# Autodesk Inventor assembly: Draft_01
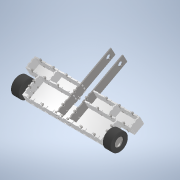
[picture p0: Inventor's stored thumbnail of the model, 180x180]
Saved by Autodesk Inventor 2021 (Build 250183000, 183)
## iProperties
Created: 2021-03-05
Part Number: Draft_01
Document SubType Name: Assembly
Designer: M3rob
Mass: 48019.6 g
Surface Area: 29850.8 cm^2
Volume: 13431.3 cm^3
Density: 3.57521 g/cm^3
Author: M3rob
## Documents named in this file (13)
- C:\Users\M3rob\Documents\GrabCAD\FireBird 250 Pound Gaming Machine\Drafts\FrameDrafts\Draft_01\Draft_01.iam
- C:\Users\M3rob\Documents\GrabCAD\FireBird 250 Pound Gaming Machine\Drafts\FrameDrafts\Draft_01\BackWallFrame.ipt
- C:\Users\M3rob\Documents\GrabCAD\FireBird 250 Pound Gaming Machine\Drafts\FrameDrafts\Draft_01\DriveFrame.ipt
- C:\Users\M3rob\Documents\GrabCAD\FireBird 250 Pound Gaming Machine\Drafts\FrameDrafts\Draft_01\NeckFrame.ipt
- C:\Users\M3rob\Documents\GrabCAD\FireBird 250 Pound Gaming Machine\Drafts\FrameDrafts\Draft_01\FrontFrame.ipt
- C:\Users\M3rob\Documents\GrabCAD\FireBird 250 Pound Gaming Machine\Drafts\FrameDrafts\Draft_01\SmallSideFrame.ipt
- C:\Users\M3rob\Documents\GrabCAD\FireBird 250 Pound Gaming Machine\Drafts\FrameDrafts\Draft_01\AluminumTopPlate.ipt
- C:\Users\M3rob\Documents\Inventor\Content Center Files\R2021\en-US\AS 2465(2)\AS 2465 - 1_2 x 1 1_4  UNC.ipt
- C:\Users\M3rob\Documents\Inventor\Content Center Files\R2021\en-US\AS 2465(1)\AS 2465 - 1_2  UNC(1).ipt
- C:\Users\M3rob\Documents\GrabCAD\FireBird 250 Pound Gaming Machine\Drafts\FrameDrafts\Draft_01\WheelDraft.ipt
- C:\Users\M3rob\Documents\CAD Add\Free Surface Imperfections\Smudges_02.png
- C:\Users\M3rob\Documents\CAD Add\Free Surface Imperfections\Scratches_03.png
- C:\Users\M3rob\Documents\CAD Add\Free Surface Imperfections\Scratches_06.png
## Components (125 placed, 9 different names)
1. BackWallFrame:1 — Flush:1, Mate:1, Mate:2, Mate:3, Mate:4, Flush:2, Mate:5, Mate:6, Mate:7, Mate:8, Mate:9, Mate:10, Mate:37, Mate:258
2. DriveFrame:1 — Mate:3, Mate:4, Flush:2, Mate:254, Mate:257
3. DriveFrame:2 — Flush:1, Mate:1, Mate:2, Mate:13, Mate:255, Mate:256
4. NeckFrame:1 — Mate:5, Mate:6, Mate:7, Mate:11, Mate:12, Mate:14, Mate:15, Mate:16
5. NeckFrame:2 — Mate:8, Mate:9, Mate:10, Mate:17, Mate:18, Mate:19, Mate:20, Mate:21, Mate:22, Mate:36, Angle:1
6. FrontFrame:1 — Mate:11, Mate:12, Mate:16, Mate:24, Mate:25, Mate:26, Mate:27, Mate:28
7. FrontFrame:2 — Mate:20, Mate:21, Mate:22, Mate:29, Mate:32, Mate:34, Mate:35, Mate:93, Mate:95, Mate:97, Mate:99, Mate:101, Mate:103, Mate:105, Mate:107, Mate:109, Mate:111, Mate:113, Mate:115, Mate:117, Mate:119, Mate:121, Mate:123, Mate:125, Mate:127, Mate:129, Mate:131, Mate:133, Mate:135, Mate:137, Mate:139, Mate:141, Mate:143, Mate:145
8. FrontFrame:3 — Mate:13, Mate:14, Mate:15, Mate:23
9. FrontFrame:4 — Mate:17, Mate:18, Mate:19, Mate:30, Mate:31, Mate:33, Flush:4, Flush:6, Mate:201, Mate:203, Mate:205, Mate:207, Mate:209, Mate:211, Mate:213, Mate:215, Mate:217, Mate:219, Mate:221, Mate:223, Mate:225, Mate:227, Mate:229, Mate:231, Mate:233, Mate:235, Mate:237, Mate:239, Mate:241, Mate:243, Mate:245, Mate:247, Mate:249, Mate:251, Mate:253
10. SmallSideFrame:1 — Mate:23, Mate:24, Mate:25
11. SmallSideFrame:2 — Mate:26, Mate:27, Mate:28
12. SmallSideFrame:3 — Mate:32, Mate:33, Mate:34, Mate:35
13. SmallSideFrame:4 — Mate:29, Mate:30, Mate:31, Flush:7, Flush:8
14. AluminumTopPlate:1 — Mate:37, Flush:6, Flush:7, Mate:38, Mate:39, Mate:40, Mate:41, Mate:42, Mate:43, Mate:44, Mate:45, Mate:46, Mate:47, Mate:48, Mate:49, Mate:50, Mate:51, Mate:52, Mate:53, Mate:54, Mate:55, Mate:56, Mate:57, Mate:58, Mate:59, Mate:60, Mate:61, Mate:62, Mate:63, Mate:64, Mate:65, Mate:66, Mate:67, Mate:68, Mate:69, Mate:70, Mate:71, Mate:72, Mate:73, Mate:74, Mate:75, Mate:76, Mate:77, Mate:78, Mate:79, Mate:80, Mate:81, Mate:82, Mate:83, Mate:84, Mate:85, Mate:86, Mate:87, Mate:88, Mate:89, Mate:90, Mate:91, Mate:92, Mate:94, Mate:96, Mate:98, Mate:100, Mate:102, Mate:104, Mate:106, Mate:108, Mate:110, Mate:112, Mate:114, Mate:116, Mate:118, Mate:120, Mate:122, Mate:124, Mate:126, Mate:128, Mate:130, Mate:132, Mate:134, Mate:136, Mate:138, Mate:140, Mate:142, Mate:144
15. AluminumTopPlate:2 — Flush:4, Mate:36, Mate:146, Mate:147, Mate:148, Mate:149, Mate:150, Mate:151, Mate:152, Mate:153, Mate:154, Mate:155, Mate:156, Mate:157, Mate:158, Mate:159, Mate:160, Mate:161, Mate:162, Mate:163, Mate:164, Mate:165, Mate:166, Mate:167, Mate:168, Mate:169, Mate:170, Mate:171, Mate:172, Mate:173, Mate:174, Mate:175, Mate:176, Mate:177, Mate:178, Mate:179, Mate:180, Mate:181, Mate:182, Mate:183, Mate:184, Mate:185, Mate:186, Mate:187, Mate:188, Mate:189, Mate:190, Mate:191, Mate:192, Mate:193, Mate:194, Mate:195, Mate:196, Mate:197, Mate:198, Mate:199, Mate:200, Mate:202, Mate:204, Mate:206, Mate:208, Mate:210, Mate:212, Mate:214, Mate:216, Mate:218, Mate:220, Mate:222, Mate:224, Mate:226, Mate:228, Mate:230, Mate:232, Mate:234, Mate:236, Mate:238, Mate:240, Mate:242, Mate:244, Mate:246, Mate:248, Mate:250, Mate:252, Flush:8
16. AS 2465 - Inch 1/2 x 1 1/4  UNC:1 — Mate:38, Mate:39
17. AS 2465 - Inch 1/2  UNC:1 — Mate:92, Mate:93
18. AS 2465 - Inch 1/2 x 1 1/4  UNC:2 — Mate:40, Mate:41
19. AS 2465 - Inch 1/2 x 1 1/4  UNC:3 — Mate:42, Mate:43
20. AS 2465 - Inch 1/2 x 1 1/4  UNC:4 — Mate:44, Mate:45
21. AS 2465 - Inch 1/2 x 1 1/4  UNC:5 — Mate:46, Mate:47
22. AS 2465 - Inch 1/2 x 1 1/4  UNC:6 — Mate:48, Mate:49
23. AS 2465 - Inch 1/2 x 1 1/4  UNC:7 — Mate:50, Mate:51
24. AS 2465 - Inch 1/2 x 1 1/4  UNC:8 — Mate:52, Mate:53
25. AS 2465 - Inch 1/2 x 1 1/4  UNC:9 — Mate:54, Mate:55
26. AS 2465 - Inch 1/2 x 1 1/4  UNC:10 — Mate:56, Mate:57
27. AS 2465 - Inch 1/2 x 1 1/4  UNC:11 — Mate:58, Mate:59
28. AS 2465 - Inch 1/2 x 1 1/4  UNC:12 — Mate:60, Mate:61
29. AS 2465 - Inch 1/2 x 1 1/4  UNC:13 — Mate:62, Mate:63
30. AS 2465 - Inch 1/2 x 1 1/4  UNC:14 — Mate:64, Mate:65
31. AS 2465 - Inch 1/2 x 1 1/4  UNC:15 — Mate:66, Mate:67
32. AS 2465 - Inch 1/2 x 1 1/4  UNC:16 — Mate:68, Mate:69
33. AS 2465 - Inch 1/2 x 1 1/4  UNC:17 — Mate:70, Mate:71
34. AS 2465 - Inch 1/2 x 1 1/4  UNC:18 — Mate:72, Mate:73
35. AS 2465 - Inch 1/2 x 1 1/4  UNC:19 — Mate:74, Mate:75
36. AS 2465 - Inch 1/2 x 1 1/4  UNC:20 — Mate:76, Mate:77
37. AS 2465 - Inch 1/2 x 1 1/4  UNC:21 — Mate:78, Mate:79
38. AS 2465 - Inch 1/2 x 1 1/4  UNC:22 — Mate:80, Mate:81
39. AS 2465 - Inch 1/2 x 1 1/4  UNC:23 — Mate:82, Mate:83
40. AS 2465 - Inch 1/2 x 1 1/4  UNC:24 — Mate:84, Mate:85
41. AS 2465 - Inch 1/2 x 1 1/4  UNC:25 — Mate:86, Mate:87
42. AS 2465 - Inch 1/2 x 1 1/4  UNC:26 — Mate:88, Mate:89
43. AS 2465 - Inch 1/2 x 1 1/4  UNC:27 — Mate:90, Mate:91
44. AS 2465 - Inch 1/2  UNC:2 — Mate:94, Mate:95
45. AS 2465 - Inch 1/2  UNC:3 — Mate:96, Mate:97
46. AS 2465 - Inch 1/2  UNC:4 — Mate:98, Mate:99
47. AS 2465 - Inch 1/2  UNC:5 — Mate:100, Mate:101
48. AS 2465 - Inch 1/2  UNC:6 — Mate:102, Mate:103
49. AS 2465 - Inch 1/2  UNC:7 — Mate:104, Mate:105
50. AS 2465 - Inch 1/2  UNC:8 — Mate:106, Mate:107
51. AS 2465 - Inch 1/2  UNC:9 — Mate:108, Mate:109
52. AS 2465 - Inch 1/2  UNC:10 — Mate:110, Mate:111
53. AS 2465 - Inch 1/2  UNC:11 — Mate:112, Mate:113
54. AS 2465 - Inch 1/2  UNC:12 — Mate:114, Mate:115
55. AS 2465 - Inch 1/2  UNC:13 — Mate:116, Mate:117
56. AS 2465 - Inch 1/2  UNC:14 — Mate:118, Mate:119
57. AS 2465 - Inch 1/2  UNC:15 — Mate:120, Mate:121
58. AS 2465 - Inch 1/2  UNC:16 — Mate:122, Mate:123
59. AS 2465 - Inch 1/2  UNC:17 — Mate:124, Mate:125
60. AS 2465 - Inch 1/2  UNC:18 — Mate:126, Mate:127
61. AS 2465 - Inch 1/2  UNC:19 — Mate:128, Mate:129
62. AS 2465 - Inch 1/2  UNC:20 — Mate:130, Mate:131
63. AS 2465 - Inch 1/2  UNC:21 — Mate:132, Mate:133
64. AS 2465 - Inch 1/2  UNC:22 — Mate:134, Mate:135
65. AS 2465 - Inch 1/2  UNC:23 — Mate:136, Mate:137
66. AS 2465 - Inch 1/2  UNC:24 — Mate:138, Mate:139
67. AS 2465 - Inch 1/2  UNC:25 — Mate:140, Mate:141
68. AS 2465 - Inch 1/2  UNC:26 — Mate:142, Mate:143
69. AS 2465 - Inch 1/2  UNC:27 — Mate:144, Mate:145
70. AS 2465 - Inch 1/2 x 1 1/4  UNC:28 — Mate:146, Mate:147
71. AS 2465 - Inch 1/2  UNC:28 — Mate:200, Mate:201
72. AS 2465 - Inch 1/2 x 1 1/4  UNC:29 — Mate:148, Mate:149
73. AS 2465 - Inch 1/2 x 1 1/4  UNC:30 — Mate:150, Mate:151
74. AS 2465 - Inch 1/2 x 1 1/4  UNC:31 — Mate:152, Mate:153
75. AS 2465 - Inch 1/2 x 1 1/4  UNC:32 — Mate:154, Mate:155
76. AS 2465 - Inch 1/2 x 1 1/4  UNC:33 — Mate:156, Mate:157
77. AS 2465 - Inch 1/2 x 1 1/4  UNC:34 — Mate:158, Mate:159
78. AS 2465 - Inch 1/2 x 1 1/4  UNC:35 — Mate:160, Mate:161
79. AS 2465 - Inch 1/2 x 1 1/4  UNC:36 — Mate:162, Mate:163
80. AS 2465 - Inch 1/2 x 1 1/4  UNC:37 — Mate:164, Mate:165
81. AS 2465 - Inch 1/2 x 1 1/4  UNC:38 — Mate:166, Mate:167
82. AS 2465 - Inch 1/2 x 1 1/4  UNC:39 — Mate:168, Mate:169
83. AS 2465 - Inch 1/2 x 1 1/4  UNC:40 — Mate:170, Mate:171
84. AS 2465 - Inch 1/2 x 1 1/4  UNC:41 — Mate:172, Mate:173
85. AS 2465 - Inch 1/2 x 1 1/4  UNC:42 — Mate:174, Mate:175
86. AS 2465 - Inch 1/2 x 1 1/4  UNC:43 — Mate:176, Mate:177
87. AS 2465 - Inch 1/2 x 1 1/4  UNC:44 — Mate:178, Mate:179
88. AS 2465 - Inch 1/2 x 1 1/4  UNC:45 — Mate:180, Mate:181
89. AS 2465 - Inch 1/2 x 1 1/4  UNC:46 — Mate:182, Mate:183
90. AS 2465 - Inch 1/2 x 1 1/4  UNC:47 — Mate:184, Mate:185
91. AS 2465 - Inch 1/2 x 1 1/4  UNC:48 — Mate:186, Mate:187
92. AS 2465 - Inch 1/2 x 1 1/4  UNC:49 — Mate:188, Mate:189
93. AS 2465 - Inch 1/2 x 1 1/4  UNC:50 — Mate:190, Mate:191
94. AS 2465 - Inch 1/2 x 1 1/4  UNC:51 — Mate:192, Mate:193
95. AS 2465 - Inch 1/2 x 1 1/4  UNC:52 — Mate:194, Mate:195
96. AS 2465 - Inch 1/2 x 1 1/4  UNC:53 — Mate:196, Mate:197
97. AS 2465 - Inch 1/2 x 1 1/4  UNC:54 — Mate:198, Mate:199
98. AS 2465 - Inch 1/2  UNC:29 — Mate:202, Mate:203
99. AS 2465 - Inch 1/2  UNC:30 — Mate:204, Mate:205
100. AS 2465 - Inch 1/2  UNC:31 — Mate:206, Mate:207
101. AS 2465 - Inch 1/2  UNC:32 — Mate:208, Mate:209
102. AS 2465 - Inch 1/2  UNC:33 — Mate:210, Mate:211
103. AS 2465 - Inch 1/2  UNC:34 — Mate:212, Mate:213
104. AS 2465 - Inch 1/2  UNC:35 — Mate:214, Mate:215
105. AS 2465 - Inch 1/2  UNC:36 — Mate:216, Mate:217
106. AS 2465 - Inch 1/2  UNC:37 — Mate:218, Mate:219
107. AS 2465 - Inch 1/2  UNC:38 — Mate:220, Mate:221
108. AS 2465 - Inch 1/2  UNC:39 — Mate:222, Mate:223
109. AS 2465 - Inch 1/2  UNC:40 — Mate:224, Mate:225
110. AS 2465 - Inch 1/2  UNC:41 — Mate:226, Mate:227
111. AS 2465 - Inch 1/2  UNC:42 — Mate:228, Mate:229
112. AS 2465 - Inch 1/2  UNC:43 — Mate:230, Mate:231
113. AS 2465 - Inch 1/2  UNC:44 — Mate:232, Mate:233
114. AS 2465 - Inch 1/2  UNC:45 — Mate:234, Mate:235
115. AS 2465 - Inch 1/2  UNC:46 — Mate:236, Mate:237
116. AS 2465 - Inch 1/2  UNC:47 — Mate:238, Mate:239
117. AS 2465 - Inch 1/2  UNC:48 — Mate:240, Mate:241
118. AS 2465 - Inch 1/2  UNC:49 — Mate:242, Mate:243
119. AS 2465 - Inch 1/2  UNC:50 — Mate:244, Mate:245
120. AS 2465 - Inch 1/2  UNC:51 — Mate:246, Mate:247
121. AS 2465 - Inch 1/2  UNC:52 — Mate:248, Mate:249
122. AS 2465 - Inch 1/2  UNC:53 — Mate:250, Mate:251
123. AS 2465 - Inch 1/2  UNC:54 — Mate:252, Mate:253
124. WheelDraft:1 — Mate:254, Mate:257
125. WheelDraft:2 — Mate:255, Mate:256
## Relationships (265: Mate 258, Flush 6, Angle 1)
- Flush:1: BackWallFrame:1 ↔ DriveFrame:2
- Mate:1: BackWallFrame:1 ↔ DriveFrame:2
- Mate:2: BackWallFrame:1 ↔ DriveFrame:2
- Mate:3: BackWallFrame:1 ↔ DriveFrame:1
- Mate:4: BackWallFrame:1 ↔ DriveFrame:1
- Flush:2: BackWallFrame:1 ↔ DriveFrame:1
- Mate:5: BackWallFrame:1 ↔ NeckFrame:1
- Mate:6: BackWallFrame:1 ↔ NeckFrame:1
- Mate:7: BackWallFrame:1 ↔ NeckFrame:1
- Mate:8: BackWallFrame:1 ↔ NeckFrame:2
- Mate:9: BackWallFrame:1 ↔ NeckFrame:2
- Mate:10: BackWallFrame:1 ↔ NeckFrame:2
- Mate:11: NeckFrame:1 ↔ FrontFrame:1
- Mate:12: NeckFrame:1 ↔ FrontFrame:1
- Mate:13: DriveFrame:2 ↔ FrontFrame:3
- Mate:14: NeckFrame:1 ↔ FrontFrame:3
- Mate:15: NeckFrame:1 ↔ FrontFrame:3
- Mate:16: NeckFrame:1 ↔ FrontFrame:1
- Mate:17: NeckFrame:2 ↔ FrontFrame:4
- Mate:18: NeckFrame:2 ↔ FrontFrame:4
- Mate:19: NeckFrame:2 ↔ FrontFrame:4
- Mate:20: NeckFrame:2 ↔ FrontFrame:2
- Mate:21: NeckFrame:2 ↔ FrontFrame:2
- Mate:22: NeckFrame:2 ↔ FrontFrame:2
- Mate:23: FrontFrame:3 ↔ SmallSideFrame:1
- Mate:24: FrontFrame:1 ↔ SmallSideFrame:1
- Mate:25: FrontFrame:1 ↔ SmallSideFrame:1
- Mate:26: FrontFrame:1 ↔ SmallSideFrame:2
- Mate:27: FrontFrame:1 ↔ SmallSideFrame:2
- Mate:28: FrontFrame:1 ↔ SmallSideFrame:2
- Mate:29: FrontFrame:2 ↔ SmallSideFrame:4
- Mate:30: FrontFrame:4 ↔ SmallSideFrame:4
- Mate:31: FrontFrame:4 ↔ SmallSideFrame:4
- Mate:32: FrontFrame:2 ↔ SmallSideFrame:3
- Mate:33: FrontFrame:4 ↔ SmallSideFrame:3
- Mate:34: FrontFrame:2 ↔ SmallSideFrame:3
- Mate:35: FrontFrame:2 ↔ SmallSideFrame:3
- Flush:4: FrontFrame:4 ↔ AluminumTopPlate:2
- Mate:36: NeckFrame:2 ↔ AluminumTopPlate:2
- Mate:37: BackWallFrame:1 ↔ AluminumTopPlate:1
- Flush:6: FrontFrame:4 ↔ AluminumTopPlate:1
- Flush:7: SmallSideFrame:4 ↔ AluminumTopPlate:1
- Mate:38: AluminumTopPlate:1 ↔ AS 2465 - Inch 1/2 x 1 1/4  UNC:1
- Mate:39: AluminumTopPlate:1 ↔ AS 2465 - Inch 1/2 x 1 1/4  UNC:1
- Mate:40: AluminumTopPlate:1 ↔ AS 2465 - Inch 1/2 x 1 1/4  UNC:2
- Mate:41: AluminumTopPlate:1 ↔ AS 2465 - Inch 1/2 x 1 1/4  UNC:2
- Mate:42: AluminumTopPlate:1 ↔ AS 2465 - Inch 1/2 x 1 1/4  UNC:3
- Mate:43: AluminumTopPlate:1 ↔ AS 2465 - Inch 1/2 x 1 1/4  UNC:3
- Mate:44: AluminumTopPlate:1 ↔ AS 2465 - Inch 1/2 x 1 1/4  UNC:4
- Mate:45: AluminumTopPlate:1 ↔ AS 2465 - Inch 1/2 x 1 1/4  UNC:4
- Mate:46: AluminumTopPlate:1 ↔ AS 2465 - Inch 1/2 x 1 1/4  UNC:5
- Mate:47: AluminumTopPlate:1 ↔ AS 2465 - Inch 1/2 x 1 1/4  UNC:5
- Mate:48: AluminumTopPlate:1 ↔ AS 2465 - Inch 1/2 x 1 1/4  UNC:6
- Mate:49: AluminumTopPlate:1 ↔ AS 2465 - Inch 1/2 x 1 1/4  UNC:6
- Mate:50: AluminumTopPlate:1 ↔ AS 2465 - Inch 1/2 x 1 1/4  UNC:7
- Mate:51: AluminumTopPlate:1 ↔ AS 2465 - Inch 1/2 x 1 1/4  UNC:7
- Mate:52: AluminumTopPlate:1 ↔ AS 2465 - Inch 1/2 x 1 1/4  UNC:8
- Mate:53: AluminumTopPlate:1 ↔ AS 2465 - Inch 1/2 x 1 1/4  UNC:8
- Mate:54: AluminumTopPlate:1 ↔ AS 2465 - Inch 1/2 x 1 1/4  UNC:9
- Mate:55: AluminumTopPlate:1 ↔ AS 2465 - Inch 1/2 x 1 1/4  UNC:9
- Mate:56: AluminumTopPlate:1 ↔ AS 2465 - Inch 1/2 x 1 1/4  UNC:10
- Mate:57: AluminumTopPlate:1 ↔ AS 2465 - Inch 1/2 x 1 1/4  UNC:10
- Mate:58: AluminumTopPlate:1 ↔ AS 2465 - Inch 1/2 x 1 1/4  UNC:11
- Mate:59: AluminumTopPlate:1 ↔ AS 2465 - Inch 1/2 x 1 1/4  UNC:11
- Mate:60: AluminumTopPlate:1 ↔ AS 2465 - Inch 1/2 x 1 1/4  UNC:12
- Mate:61: AluminumTopPlate:1 ↔ AS 2465 - Inch 1/2 x 1 1/4  UNC:12
- Mate:62: AluminumTopPlate:1 ↔ AS 2465 - Inch 1/2 x 1 1/4  UNC:13
- Mate:63: AluminumTopPlate:1 ↔ AS 2465 - Inch 1/2 x 1 1/4  UNC:13
- Mate:64: AluminumTopPlate:1 ↔ AS 2465 - Inch 1/2 x 1 1/4  UNC:14
- Mate:65: AluminumTopPlate:1 ↔ AS 2465 - Inch 1/2 x 1 1/4  UNC:14
- Mate:66: AluminumTopPlate:1 ↔ AS 2465 - Inch 1/2 x 1 1/4  UNC:15
- Mate:67: AluminumTopPlate:1 ↔ AS 2465 - Inch 1/2 x 1 1/4  UNC:15
- Mate:68: AluminumTopPlate:1 ↔ AS 2465 - Inch 1/2 x 1 1/4  UNC:16
- Mate:69: AluminumTopPlate:1 ↔ AS 2465 - Inch 1/2 x 1 1/4  UNC:16
- Mate:70: AluminumTopPlate:1 ↔ AS 2465 - Inch 1/2 x 1 1/4  UNC:17
- Mate:71: AluminumTopPlate:1 ↔ AS 2465 - Inch 1/2 x 1 1/4  UNC:17
- Mate:72: AluminumTopPlate:1 ↔ AS 2465 - Inch 1/2 x 1 1/4  UNC:18
- Mate:73: AluminumTopPlate:1 ↔ AS 2465 - Inch 1/2 x 1 1/4  UNC:18
- Mate:74: AluminumTopPlate:1 ↔ AS 2465 - Inch 1/2 x 1 1/4  UNC:19
- Mate:75: AluminumTopPlate:1 ↔ AS 2465 - Inch 1/2 x 1 1/4  UNC:19
- Mate:76: AluminumTopPlate:1 ↔ AS 2465 - Inch 1/2 x 1 1/4  UNC:20
- Mate:77: AluminumTopPlate:1 ↔ AS 2465 - Inch 1/2 x 1 1/4  UNC:20
- Mate:78: AluminumTopPlate:1 ↔ AS 2465 - Inch 1/2 x 1 1/4  UNC:21
- Mate:79: AluminumTopPlate:1 ↔ AS 2465 - Inch 1/2 x 1 1/4  UNC:21
- Mate:80: AluminumTopPlate:1 ↔ AS 2465 - Inch 1/2 x 1 1/4  UNC:22
- Mate:81: AluminumTopPlate:1 ↔ AS 2465 - Inch 1/2 x 1 1/4  UNC:22
- Mate:82: AluminumTopPlate:1 ↔ AS 2465 - Inch 1/2 x 1 1/4  UNC:23
- Mate:83: AluminumTopPlate:1 ↔ AS 2465 - Inch 1/2 x 1 1/4  UNC:23
- Mate:84: AluminumTopPlate:1 ↔ AS 2465 - Inch 1/2 x 1 1/4  UNC:24
- Mate:85: AluminumTopPlate:1 ↔ AS 2465 - Inch 1/2 x 1 1/4  UNC:24
- Mate:86: AluminumTopPlate:1 ↔ AS 2465 - Inch 1/2 x 1 1/4  UNC:25
- Mate:87: AluminumTopPlate:1 ↔ AS 2465 - Inch 1/2 x 1 1/4  UNC:25
- Mate:88: AluminumTopPlate:1 ↔ AS 2465 - Inch 1/2 x 1 1/4  UNC:26
- Mate:89: AluminumTopPlate:1 ↔ AS 2465 - Inch 1/2 x 1 1/4  UNC:26
- Mate:90: AluminumTopPlate:1 ↔ AS 2465 - Inch 1/2 x 1 1/4  UNC:27
- Mate:91: AluminumTopPlate:1 ↔ AS 2465 - Inch 1/2 x 1 1/4  UNC:27
- Mate:92: AluminumTopPlate:1 ↔ AS 2465 - Inch 1/2  UNC:1
- Mate:93: FrontFrame:2 ↔ AS 2465 - Inch 1/2  UNC:1
- Mate:94: AluminumTopPlate:1 ↔ AS 2465 - Inch 1/2  UNC:2
- Mate:95: FrontFrame:2 ↔ AS 2465 - Inch 1/2  UNC:2
- Mate:96: AluminumTopPlate:1 ↔ AS 2465 - Inch 1/2  UNC:3
- Mate:97: FrontFrame:2 ↔ AS 2465 - Inch 1/2  UNC:3
- Mate:98: AluminumTopPlate:1 ↔ AS 2465 - Inch 1/2  UNC:4
- Mate:99: FrontFrame:2 ↔ AS 2465 - Inch 1/2  UNC:4
- Mate:100: AluminumTopPlate:1 ↔ AS 2465 - Inch 1/2  UNC:5
- Mate:101: FrontFrame:2 ↔ AS 2465 - Inch 1/2  UNC:5
- Mate:102: AluminumTopPlate:1 ↔ AS 2465 - Inch 1/2  UNC:6
- Mate:103: FrontFrame:2 ↔ AS 2465 - Inch 1/2  UNC:6
- Mate:104: AluminumTopPlate:1 ↔ AS 2465 - Inch 1/2  UNC:7
- Mate:105: FrontFrame:2 ↔ AS 2465 - Inch 1/2  UNC:7
- Mate:106: AluminumTopPlate:1 ↔ AS 2465 - Inch 1/2  UNC:8
- Mate:107: FrontFrame:2 ↔ AS 2465 - Inch 1/2  UNC:8
- Mate:108: AluminumTopPlate:1 ↔ AS 2465 - Inch 1/2  UNC:9
- Mate:109: FrontFrame:2 ↔ AS 2465 - Inch 1/2  UNC:9
- Mate:110: AluminumTopPlate:1 ↔ AS 2465 - Inch 1/2  UNC:10
- Mate:111: FrontFrame:2 ↔ AS 2465 - Inch 1/2  UNC:10
- Mate:112: AluminumTopPlate:1 ↔ AS 2465 - Inch 1/2  UNC:11
- Mate:113: FrontFrame:2 ↔ AS 2465 - Inch 1/2  UNC:11
- Mate:114: AluminumTopPlate:1 ↔ AS 2465 - Inch 1/2  UNC:12
- Mate:115: FrontFrame:2 ↔ AS 2465 - Inch 1/2  UNC:12
- Mate:116: AluminumTopPlate:1 ↔ AS 2465 - Inch 1/2  UNC:13
- Mate:117: FrontFrame:2 ↔ AS 2465 - Inch 1/2  UNC:13
- Mate:118: AluminumTopPlate:1 ↔ AS 2465 - Inch 1/2  UNC:14
- Mate:119: FrontFrame:2 ↔ AS 2465 - Inch 1/2  UNC:14
- Mate:120: AluminumTopPlate:1 ↔ AS 2465 - Inch 1/2  UNC:15
- Mate:121: FrontFrame:2 ↔ AS 2465 - Inch 1/2  UNC:15
- Mate:122: AluminumTopPlate:1 ↔ AS 2465 - Inch 1/2  UNC:16
- Mate:123: FrontFrame:2 ↔ AS 2465 - Inch 1/2  UNC:16
- Mate:124: AluminumTopPlate:1 ↔ AS 2465 - Inch 1/2  UNC:17
- Mate:125: FrontFrame:2 ↔ AS 2465 - Inch 1/2  UNC:17
- Mate:126: AluminumTopPlate:1 ↔ AS 2465 - Inch 1/2  UNC:18
- Mate:127: FrontFrame:2 ↔ AS 2465 - Inch 1/2  UNC:18
- Mate:128: AluminumTopPlate:1 ↔ AS 2465 - Inch 1/2  UNC:19
- Mate:129: FrontFrame:2 ↔ AS 2465 - Inch 1/2  UNC:19
- Mate:130: AluminumTopPlate:1 ↔ AS 2465 - Inch 1/2  UNC:20
- Mate:131: FrontFrame:2 ↔ AS 2465 - Inch 1/2  UNC:20
- Mate:132: AluminumTopPlate:1 ↔ AS 2465 - Inch 1/2  UNC:21
- Mate:133: FrontFrame:2 ↔ AS 2465 - Inch 1/2  UNC:21
- Mate:134: AluminumTopPlate:1 ↔ AS 2465 - Inch 1/2  UNC:22
- Mate:135: FrontFrame:2 ↔ AS 2465 - Inch 1/2  UNC:22
- Mate:136: AluminumTopPlate:1 ↔ AS 2465 - Inch 1/2  UNC:23
- Mate:137: FrontFrame:2 ↔ AS 2465 - Inch 1/2  UNC:23
- Mate:138: AluminumTopPlate:1 ↔ AS 2465 - Inch 1/2  UNC:24
- Mate:139: FrontFrame:2 ↔ AS 2465 - Inch 1/2  UNC:24
- Mate:140: AluminumTopPlate:1 ↔ AS 2465 - Inch 1/2  UNC:25
- Mate:141: FrontFrame:2 ↔ AS 2465 - Inch 1/2  UNC:25
- Mate:142: AluminumTopPlate:1 ↔ AS 2465 - Inch 1/2  UNC:26
- Mate:143: FrontFrame:2 ↔ AS 2465 - Inch 1/2  UNC:26
- Mate:144: AluminumTopPlate:1 ↔ AS 2465 - Inch 1/2  UNC:27
- Mate:145: FrontFrame:2 ↔ AS 2465 - Inch 1/2  UNC:27
- Mate:146: AluminumTopPlate:2 ↔ AS 2465 - Inch 1/2 x 1 1/4  UNC:28
- Mate:147: AluminumTopPlate:2 ↔ AS 2465 - Inch 1/2 x 1 1/4  UNC:28
- Mate:148: AluminumTopPlate:2 ↔ AS 2465 - Inch 1/2 x 1 1/4  UNC:29
- Mate:149: AluminumTopPlate:2 ↔ AS 2465 - Inch 1/2 x 1 1/4  UNC:29
- Mate:150: AluminumTopPlate:2 ↔ AS 2465 - Inch 1/2 x 1 1/4  UNC:30
- Mate:151: AluminumTopPlate:2 ↔ AS 2465 - Inch 1/2 x 1 1/4  UNC:30
- Mate:152: AluminumTopPlate:2 ↔ AS 2465 - Inch 1/2 x 1 1/4  UNC:31
- Mate:153: AluminumTopPlate:2 ↔ AS 2465 - Inch 1/2 x 1 1/4  UNC:31
- Mate:154: AluminumTopPlate:2 ↔ AS 2465 - Inch 1/2 x 1 1/4  UNC:32
- Mate:155: AluminumTopPlate:2 ↔ AS 2465 - Inch 1/2 x 1 1/4  UNC:32
- Mate:156: AluminumTopPlate:2 ↔ AS 2465 - Inch 1/2 x 1 1/4  UNC:33
- Mate:157: AluminumTopPlate:2 ↔ AS 2465 - Inch 1/2 x 1 1/4  UNC:33
- Mate:158: AluminumTopPlate:2 ↔ AS 2465 - Inch 1/2 x 1 1/4  UNC:34
- Mate:159: AluminumTopPlate:2 ↔ AS 2465 - Inch 1/2 x 1 1/4  UNC:34
- Mate:160: AluminumTopPlate:2 ↔ AS 2465 - Inch 1/2 x 1 1/4  UNC:35
- Mate:161: AluminumTopPlate:2 ↔ AS 2465 - Inch 1/2 x 1 1/4  UNC:35
- Mate:162: AluminumTopPlate:2 ↔ AS 2465 - Inch 1/2 x 1 1/4  UNC:36
- Mate:163: AluminumTopPlate:2 ↔ AS 2465 - Inch 1/2 x 1 1/4  UNC:36
- Mate:164: AluminumTopPlate:2 ↔ AS 2465 - Inch 1/2 x 1 1/4  UNC:37
- Mate:165: AluminumTopPlate:2 ↔ AS 2465 - Inch 1/2 x 1 1/4  UNC:37
- Mate:166: AluminumTopPlate:2 ↔ AS 2465 - Inch 1/2 x 1 1/4  UNC:38
- Mate:167: AluminumTopPlate:2 ↔ AS 2465 - Inch 1/2 x 1 1/4  UNC:38
- Mate:168: AluminumTopPlate:2 ↔ AS 2465 - Inch 1/2 x 1 1/4  UNC:39
- Mate:169: AluminumTopPlate:2 ↔ AS 2465 - Inch 1/2 x 1 1/4  UNC:39
- Mate:170: AluminumTopPlate:2 ↔ AS 2465 - Inch 1/2 x 1 1/4  UNC:40
- Mate:171: AluminumTopPlate:2 ↔ AS 2465 - Inch 1/2 x 1 1/4  UNC:40
- Mate:172: AluminumTopPlate:2 ↔ AS 2465 - Inch 1/2 x 1 1/4  UNC:41
- Mate:173: AluminumTopPlate:2 ↔ AS 2465 - Inch 1/2 x 1 1/4  UNC:41
- Mate:174: AluminumTopPlate:2 ↔ AS 2465 - Inch 1/2 x 1 1/4  UNC:42
- Mate:175: AluminumTopPlate:2 ↔ AS 2465 - Inch 1/2 x 1 1/4  UNC:42
- Mate:176: AluminumTopPlate:2 ↔ AS 2465 - Inch 1/2 x 1 1/4  UNC:43
- Mate:177: AluminumTopPlate:2 ↔ AS 2465 - Inch 1/2 x 1 1/4  UNC:43
- Mate:178: AluminumTopPlate:2 ↔ AS 2465 - Inch 1/2 x 1 1/4  UNC:44
- Mate:179: AluminumTopPlate:2 ↔ AS 2465 - Inch 1/2 x 1 1/4  UNC:44
- Mate:180: AluminumTopPlate:2 ↔ AS 2465 - Inch 1/2 x 1 1/4  UNC:45
- Mate:181: AluminumTopPlate:2 ↔ AS 2465 - Inch 1/2 x 1 1/4  UNC:45
- Mate:182: AluminumTopPlate:2 ↔ AS 2465 - Inch 1/2 x 1 1/4  UNC:46
- Mate:183: AluminumTopPlate:2 ↔ AS 2465 - Inch 1/2 x 1 1/4  UNC:46
- Mate:184: AluminumTopPlate:2 ↔ AS 2465 - Inch 1/2 x 1 1/4  UNC:47
- Mate:185: AluminumTopPlate:2 ↔ AS 2465 - Inch 1/2 x 1 1/4  UNC:47
- Mate:186: AluminumTopPlate:2 ↔ AS 2465 - Inch 1/2 x 1 1/4  UNC:48
- Mate:187: AluminumTopPlate:2 ↔ AS 2465 - Inch 1/2 x 1 1/4  UNC:48
- Mate:188: AluminumTopPlate:2 ↔ AS 2465 - Inch 1/2 x 1 1/4  UNC:49
- Mate:189: AluminumTopPlate:2 ↔ AS 2465 - Inch 1/2 x 1 1/4  UNC:49
- Mate:190: AluminumTopPlate:2 ↔ AS 2465 - Inch 1/2 x 1 1/4  UNC:50
- Mate:191: AluminumTopPlate:2 ↔ AS 2465 - Inch 1/2 x 1 1/4  UNC:50
- Mate:192: AluminumTopPlate:2 ↔ AS 2465 - Inch 1/2 x 1 1/4  UNC:51
- Mate:193: AluminumTopPlate:2 ↔ AS 2465 - Inch 1/2 x 1 1/4  UNC:51
- Mate:194: AluminumTopPlate:2 ↔ AS 2465 - Inch 1/2 x 1 1/4  UNC:52
- Mate:195: AluminumTopPlate:2 ↔ AS 2465 - Inch 1/2 x 1 1/4  UNC:52
- Mate:196: AluminumTopPlate:2 ↔ AS 2465 - Inch 1/2 x 1 1/4  UNC:53
- Mate:197: AluminumTopPlate:2 ↔ AS 2465 - Inch 1/2 x 1 1/4  UNC:53
- Mate:198: AluminumTopPlate:2 ↔ AS 2465 - Inch 1/2 x 1 1/4  UNC:54
- Mate:199: AluminumTopPlate:2 ↔ AS 2465 - Inch 1/2 x 1 1/4  UNC:54
- Mate:200: AluminumTopPlate:2 ↔ AS 2465 - Inch 1/2  UNC:28
- Mate:201: FrontFrame:4 ↔ AS 2465 - Inch 1/2  UNC:28
- Mate:202: AluminumTopPlate:2 ↔ AS 2465 - Inch 1/2  UNC:29
- Mate:203: FrontFrame:4 ↔ AS 2465 - Inch 1/2  UNC:29
- Mate:204: AluminumTopPlate:2 ↔ AS 2465 - Inch 1/2  UNC:30
- Mate:205: FrontFrame:4 ↔ AS 2465 - Inch 1/2  UNC:30
- Mate:206: AluminumTopPlate:2 ↔ AS 2465 - Inch 1/2  UNC:31
- Mate:207: FrontFrame:4 ↔ AS 2465 - Inch 1/2  UNC:31
- Mate:208: AluminumTopPlate:2 ↔ AS 2465 - Inch 1/2  UNC:32
- Mate:209: FrontFrame:4 ↔ AS 2465 - Inch 1/2  UNC:32
- Mate:210: AluminumTopPlate:2 ↔ AS 2465 - Inch 1/2  UNC:33
- Mate:211: FrontFrame:4 ↔ AS 2465 - Inch 1/2  UNC:33
- Mate:212: AluminumTopPlate:2 ↔ AS 2465 - Inch 1/2  UNC:34
- Mate:213: FrontFrame:4 ↔ AS 2465 - Inch 1/2  UNC:34
- Mate:214: AluminumTopPlate:2 ↔ AS 2465 - Inch 1/2  UNC:35
- Mate:215: FrontFrame:4 ↔ AS 2465 - Inch 1/2  UNC:35
- Mate:216: AluminumTopPlate:2 ↔ AS 2465 - Inch 1/2  UNC:36
- Mate:217: FrontFrame:4 ↔ AS 2465 - Inch 1/2  UNC:36
- Mate:218: AluminumTopPlate:2 ↔ AS 2465 - Inch 1/2  UNC:37
- Mate:219: FrontFrame:4 ↔ AS 2465 - Inch 1/2  UNC:37
- Mate:220: AluminumTopPlate:2 ↔ AS 2465 - Inch 1/2  UNC:38
- Mate:221: FrontFrame:4 ↔ AS 2465 - Inch 1/2  UNC:38
- Mate:222: AluminumTopPlate:2 ↔ AS 2465 - Inch 1/2  UNC:39
- Mate:223: FrontFrame:4 ↔ AS 2465 - Inch 1/2  UNC:39
- Mate:224: AluminumTopPlate:2 ↔ AS 2465 - Inch 1/2  UNC:40
- Mate:225: FrontFrame:4 ↔ AS 2465 - Inch 1/2  UNC:40
- Mate:226: AluminumTopPlate:2 ↔ AS 2465 - Inch 1/2  UNC:41
- Mate:227: FrontFrame:4 ↔ AS 2465 - Inch 1/2  UNC:41
- Mate:228: AluminumTopPlate:2 ↔ AS 2465 - Inch 1/2  UNC:42
- Mate:229: FrontFrame:4 ↔ AS 2465 - Inch 1/2  UNC:42
- Mate:230: AluminumTopPlate:2 ↔ AS 2465 - Inch 1/2  UNC:43
- Mate:231: FrontFrame:4 ↔ AS 2465 - Inch 1/2  UNC:43
- Mate:232: AluminumTopPlate:2 ↔ AS 2465 - Inch 1/2  UNC:44
- Mate:233: FrontFrame:4 ↔ AS 2465 - Inch 1/2  UNC:44
- Mate:234: AluminumTopPlate:2 ↔ AS 2465 - Inch 1/2  UNC:45
- Mate:235: FrontFrame:4 ↔ AS 2465 - Inch 1/2  UNC:45
- Mate:236: AluminumTopPlate:2 ↔ AS 2465 - Inch 1/2  UNC:46
- Mate:237: FrontFrame:4 ↔ AS 2465 - Inch 1/2  UNC:46
- Mate:238: AluminumTopPlate:2 ↔ AS 2465 - Inch 1/2  UNC:47
- Mate:239: FrontFrame:4 ↔ AS 2465 - Inch 1/2  UNC:47
- Mate:240: AluminumTopPlate:2 ↔ AS 2465 - Inch 1/2  UNC:48
- Mate:241: FrontFrame:4 ↔ AS 2465 - Inch 1/2  UNC:48
- Mate:242: AluminumTopPlate:2 ↔ AS 2465 - Inch 1/2  UNC:49
- Mate:243: FrontFrame:4 ↔ AS 2465 - Inch 1/2  UNC:49
- Mate:244: AluminumTopPlate:2 ↔ AS 2465 - Inch 1/2  UNC:50
- Mate:245: FrontFrame:4 ↔ AS 2465 - Inch 1/2  UNC:50
- Mate:246: AluminumTopPlate:2 ↔ AS 2465 - Inch 1/2  UNC:51
- Mate:247: FrontFrame:4 ↔ AS 2465 - Inch 1/2  UNC:51
- Mate:248: AluminumTopPlate:2 ↔ AS 2465 - Inch 1/2  UNC:52
- Mate:249: FrontFrame:4 ↔ AS 2465 - Inch 1/2  UNC:52
- Mate:250: AluminumTopPlate:2 ↔ AS 2465 - Inch 1/2  UNC:53
- Mate:251: FrontFrame:4 ↔ AS 2465 - Inch 1/2  UNC:53
- Mate:252: AluminumTopPlate:2 ↔ AS 2465 - Inch 1/2  UNC:54
- Mate:253: FrontFrame:4 ↔ AS 2465 - Inch 1/2  UNC:54
- Flush:8: SmallSideFrame:4 ↔ AluminumTopPlate:2
- Mate:254: DriveFrame:1 ↔ WheelDraft:1
- Mate:255: DriveFrame:2 ↔ WheelDraft:2
- Mate:256 (25.4 mm): DriveFrame:2 ↔ WheelDraft:2
- Mate:257 (25.4 mm): DriveFrame:1 ↔ WheelDraft:1
- Angle:1 (180 deg): NeckFrame:2
- Mate:258: BackWallFrame:1
